# Autodesk Inventor assembly: wahacz_tylny_szkic
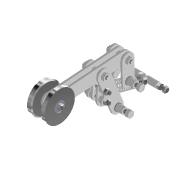
[picture p0: Inventor's stored thumbnail of the model, 180x180]
Saved by Autodesk Inventor 2020.3 (Build 243373000, 373)
## iProperties
Created: 2022-01-11
Part Number: wahacz_tylny_szkic
Document SubType Name: Assembly
Designer: patry
Author: patry
## Documents named in this file (27)
- C:\Users\patry\Desktop\Semestr 7\Inzynierka\Projekt inventor\Ariadna_inzynierka\Workspaces\Obszar roboczy\Obszar roboczy\Naped\Zawieszenie_v3\wahacz_tylny_szkic.iam
- C:\Users\patry\Desktop\Semestr 7\Inzynierka\Projekt inventor\Ariadna_inzynierka\Workspaces\Obszar roboczy\Obszar roboczy\Naped\Zawieszenie_v3\ramie_1_wahacza.ipt
- C:\Users\patry\Desktop\Semestr 7\Inzynierka\Projekt inventor\Ariadna_inzynierka\Workspaces\Obszar roboczy\Obszar roboczy\Naped\Zawieszenie_v3\tuleja_TUF106040.ipt
- C:\Users\patry\Desktop\Semestr 7\Inzynierka\Projekt inventor\Ariadna_inzynierka\Workspaces\Obszar roboczy\Obszar roboczy\Naped\Sruby\M6_nut_5mm.ipt
- C:\Users\patry\Desktop\Semestr 7\Inzynierka\Projekt inventor\Ariadna_inzynierka\Workspaces\Obszar roboczy\Obszar roboczy\Naped\Amortyzator\Korpus.ipt
- C:\Users\patry\Desktop\Semestr 7\Inzynierka\Projekt inventor\Ariadna_inzynierka\Workspaces\Obszar roboczy\Obszar roboczy\Naped\Amortyzator\Tlok.ipt
- C:\Users\patry\Desktop\Semestr 7\Inzynierka\Projekt inventor\Ariadna_inzynierka\Workspaces\Obszar roboczy\Obszar roboczy\Naped\Amortyzator\Nakretka.ipt
- C:\Users\patry\Desktop\Semestr 7\Inzynierka\Projekt inventor\Ariadna_inzynierka\Workspaces\Obszar roboczy\Obszar roboczy\Naped\Sruby\M5_nut_5mm.ipt
- C:\Users\patry\Desktop\Semestr 7\Inzynierka\Projekt inventor\Ariadna_inzynierka\Workspaces\Obszar roboczy\Obszar roboczy\Naped\Sruby\M5_70_shaft.ipt
- C:\Users\patry\Desktop\Semestr 7\Inzynierka\Projekt inventor\Ariadna_inzynierka\Workspaces\Obszar roboczy\Obszar roboczy\Naped\Sruby\M3_16_shaft.ipt
- C:\Users\patry\Desktop\Semestr 7\Inzynierka\Projekt inventor\Ariadna_inzynierka\Workspaces\Obszar roboczy\Obszar roboczy\Naped\Sruby\M3_nut_2,5mm.ipt
- C:\Users\patry\Desktop\Semestr 7\Inzynierka\Projekt inventor\Ariadna_inzynierka\Workspaces\Obszar roboczy\Obszar roboczy\Naped\Zawieszenie_v3\wspornik_amortyzatora.ipt
- C:\Users\patry\Desktop\Semestr 7\Inzynierka\Projekt inventor\Ariadna_inzynierka\Workspaces\Obszar roboczy\Obszar roboczy\Naped\Sruby\M6_40_shaft.ipt
- C:\Users\patry\Desktop\Semestr 7\Inzynierka\Projekt inventor\Ariadna_inzynierka\Workspaces\Obszar roboczy\Obszar roboczy\Naped\Sruby\tuleja_M6_M10_7.ipt
- C:\Users\patry\Desktop\Semestr 7\Inzynierka\Projekt inventor\Ariadna_inzynierka\Workspaces\Obszar roboczy\Obszar roboczy\Naped\Sruby\M6_1,25_pad.ipt
- C:\Users\patry\Desktop\Semestr 7\Inzynierka\Projekt inventor\Ariadna_inzynierka\Workspaces\Obszar roboczy\Obszar roboczy\Naped\Sruby\M6_70_shaft.ipt
- C:\Users\patry\Desktop\Semestr 7\Inzynierka\Projekt inventor\Ariadna_inzynierka\Workspaces\Obszar roboczy\Obszar roboczy\Naped\Sruby\M5_40_shaft.ipt
- M5_shaft.ipt
- C:\Users\patry\Desktop\Semestr 7\Inzynierka\Projekt inventor\Ariadna_inzynierka\Workspaces\Obszar roboczy\Obszar roboczy\Naped\Sruby\tuleja_M5_M9_4,5.ipt
- C:\Users\patry\Desktop\Semestr 7\Inzynierka\Projekt inventor\Ariadna_inzynierka\Workspaces\Obszar roboczy\Obszar roboczy\Naped\Zawieszenie_v3\glowny_wahacz_zewn.ipt
- lacznik_zewn.ipt
- C:\Users\patry\Desktop\Semestr 7\Inzynierka\Projekt inventor\Ariadna_inzynierka\Workspaces\Obszar roboczy\Obszar roboczy\Naped\Zawieszenie_v3\independent_wheel_pair.iam
- C:\Users\patry\Desktop\Semestr 7\Inzynierka\Projekt inventor\Ariadna_inzynierka\Workspaces\Obszar roboczy\Obszar roboczy\Naped\Sruby\tuleja_M6_M10_6.ipt
- C:\Users\patry\Desktop\Semestr 7\Inzynierka\Projekt inventor\Ariadna_inzynierka\Workspaces\Obszar roboczy\Obszar roboczy\Naped\Sruby\tuleja_M5_M9_17.5.ipt
- C:\Users\patry\Desktop\Semestr 7\Inzynierka\Projekt inventor\Ariadna_inzynierka\Workspaces\Obszar roboczy\Obszar roboczy\Naped\Zawieszenie_v3\ramie_2_wahacza_tylnego.ipt
- C:\Users\patry\Desktop\Semestr 7\Inzynierka\Projekt inventor\Ariadna_inzynierka\Workspaces\Obszar roboczy\Obszar roboczy\Naped\Sruby\M6x25_plaski_leb.ipt
- C:\Users\patry\Desktop\Semestr 7\Inzynierka\Projekt inventor\Ariadna_inzynierka\Workspaces\Obszar roboczy\Obszar roboczy\Naped\Zawieszenie_v3\Compress Spring11.ipt
## Components (73 placed, 24 different names)
1. ramie_1_wahacza:1
2. tuleja_TUF106040:1
3. tuleja_TUF106040:2
4. tuleja_TUF106040:3
5. tuleja_TUF106040:4
6. tuleja_TUF106040:5
7. tuleja_TUF106040:6
8. tuleja_TUF106040:7
9. tuleja_TUF106040:8
10. M6_nut_5mm:1
11. Korpus:1 — Zestawiające:139
12. Tlok:1 — Równoległe:10
13. Nakretka:1
14. M5_nut_5mm:1
15. M5_70_shaft:1
16. ramie_1_wahacza:2
17. M5_nut_5mm:2
18. M3_16_shaft:1
19. M3_nut_2,5mm:1
20. M3_nut_2,5mm:2
21. wspornik_amortyzatora:1
22. wspornik_amortyzatora:2
23. M6_40_shaft:1
24. M6_40_shaft:2
25. M6_nut_5mm:2
26. M6_nut_5mm:3
27. M6_nut_5mm:4
28. tuleja_M6_M10_7:1
29. tuleja_M6_M10_7:2
30. M6_1,25_pad:1
31. M6_1,25_pad:2
32. M6_1,25_pad:3
33. M6_1,25_pad:4
34. M6_1,25_pad:5
35. M6_1,25_pad:6
36. M6_1,25_pad:7
37. M6_1,25_pad:8
38. M6_70_shaft:1
39. M6_nut_5mm:5
40. M6_nut_5mm:6
41. M6_nut_5mm:7
42. M6_nut_5mm:8
43. M5_shaft:1
44. M5_shaft:2
45. M5_nut_5mm:3
46. M5_nut_5mm:4
47. M5_nut_5mm:5
48. M5_nut_5mm:6
49. tuleja_M5_M9_4,5:1
50. tuleja_M5_M9_4,5:2
51. tuleja_M5_M9_4,5:3
52. tuleja_M5_M9_4,5:4
53. lacznik_zewn:1
54. lacznik_zewn:2
55. independent_wheel_pair:1 [sub-assembly]
56. tuleja_M6_M10_7:3
57. tuleja_M6_M10_6:1
58. M6_nut_5mm:9
59. M6_nut_5mm:10
60. M6_nut_5mm:11
61. M6_nut_5mm:12
62. tuleja_M6_M10_6:2
63. tuleja_M6_M10_6:3
64. tuleja_M6_M10_6:4
65. M5_nut_5mm:7
66. M5_nut_5mm:8
67. tuleja_M5_M9_17.5:1
68. tuleja_M5_M9_17.5:2
69. ramie_2_wahacza_tylnego:1
70. ramie_2_wahacza_tylnego:2
71. M6x25_plaski_leb:1
72. M6x25_plaski_leb:2
73. Compress Spring1:1 — Zestawiające:139, Równoległe:10
## Relationships (152: Mate 139, Flush 10, Angle 2, CylindricalJoint 1)
- [Mate]: ramie_1_wahacza:1 ↔ tuleja_TUF106040:4
- [Mate]: ramie_1_wahacza:1 ↔ tuleja_TUF106040:4
- [Angle] (0 deg): ramie_1_wahacza:1 ↔ tuleja_TUF106040:4
- [Mate]: Korpus:1 ↔ Tlok:1
- [Angle] (0 deg): Korpus:1 ↔ Tlok:1
- [Mate]: Korpus:1 ↔ Nakretka:1
- [Mate] (10 mm): Korpus:1 ↔ Nakretka:1
- [CylindricalJoint]: Korpus:1 ↔ Tlok:1
- [Mate]: Korpus:1 ↔ M5_70_shaft:1
- [Flush] (-32.5 mm): Korpus:1 ↔ M5_70_shaft:1
- [Mate]: M5_nut_5mm:1 ↔ M5_70_shaft:1
- [Mate]: M5_70_shaft:1 ↔ M5_nut_5mm:2
- [Mate] (60 mm): M5_nut_5mm:1 ↔ M5_nut_5mm:2
- [Mate] (27.5 mm): Korpus:1 ↔ M5_nut_5mm:1
- [Mate]: tuleja_TUF106040:6 ↔ ramie_1_wahacza:2
- [Mate]: tuleja_TUF106040:5 ↔ ramie_1_wahacza:2
- [Mate]: tuleja_TUF106040:6 ↔ ramie_1_wahacza:2
- [Mate]: tuleja_TUF106040:1 ↔ tuleja_TUF106040:7
- [Mate]: wspornik_amortyzatora:1 ↔ wspornik_amortyzatora:2
- [Mate]: wspornik_amortyzatora:1 ↔ wspornik_amortyzatora:2
- [Mate] (5 mm): wspornik_amortyzatora:1 ↔ wspornik_amortyzatora:2
- [Mate]: M3_16_shaft:1 ↔ wspornik_amortyzatora:2
- [Flush] (-2.5 mm): M3_16_shaft:1 ↔ wspornik_amortyzatora:1
- [Mate]: M3_16_shaft:1 ↔ M3_nut_2,5mm:1
- [Mate]: M3_nut_2,5mm:1 ↔ wspornik_amortyzatora:1
- [Mate]: M3_16_shaft:1 ↔ M3_nut_2,5mm:2
- [Mate]: M3_nut_2,5mm:2 ↔ wspornik_amortyzatora:2
- [Mate]: Tlok:1 ↔ M3_16_shaft:1
- [Mate]: Tlok:1 ↔ wspornik_amortyzatora:2
- [Mate]: ramie_1_wahacza:1 ↔ wspornik_amortyzatora:1
- [Mate]: ramie_1_wahacza:1 ↔ wspornik_amortyzatora:1
- [Mate] (4.5 mm): ramie_1_wahacza:1 ↔ wspornik_amortyzatora:1
- [Mate]: tuleja_TUF106040:4 ↔ M6_40_shaft:1
- [Flush] (7 mm): ramie_1_wahacza:1 ↔ M6_40_shaft:1
- [Mate]: tuleja_TUF106040:7 ↔ M6_40_shaft:2
- [Mate]: M6_nut_5mm:1 ↔ M6_40_shaft:1
- [Mate]: ramie_1_wahacza:1 ↔ M6_nut_5mm:1
- [Mate]: M6_40_shaft:1 ↔ M6_nut_5mm:2
- [Mate]: ramie_1_wahacza:2 ↔ M6_nut_5mm:2
- [Mate]: M6_40_shaft:2 ↔ M6_nut_5mm:3
- [Mate]: M6_40_shaft:2 ↔ M6_nut_5mm:4
- [Mate]: M6_40_shaft:1 ↔ tuleja_M6_M10_7:1
- [Mate]: M6_40_shaft:2 ↔ tuleja_M6_M10_7:2
- [Mate]: M6_1,25_pad:1 ↔ M6_1,25_pad:2
- [Mate]: M6_1,25_pad:1 ↔ M6_1,25_pad:2
- [Mate]: M6_40_shaft:1 ↔ M6_1,25_pad:1
- [Mate]: M6_1,25_pad:3 ↔ M6_1,25_pad:4
- [Mate]: M6_1,25_pad:3 ↔ M6_1,25_pad:4
- [Mate]: M6_40_shaft:1 ↔ M6_1,25_pad:3
- [Mate]: tuleja_TUF106040:4 ↔ M6_1,25_pad:3
- [Mate]: M6_1,25_pad:5 ↔ M6_1,25_pad:6
- [Mate]: M6_1,25_pad:5 ↔ M6_1,25_pad:6
- [Mate]: M6_40_shaft:2 ↔ M6_1,25_pad:5
- [Mate]: M6_1,25_pad:7 ↔ M6_1,25_pad:8
- [Mate]: M6_1,25_pad:7 ↔ M6_1,25_pad:8
- [Mate]: M6_40_shaft:2 ↔ M6_1,25_pad:7
- [Mate]: tuleja_TUF106040:7 ↔ M6_1,25_pad:7
- [Flush]: M5_70_shaft:1 ↔ M6_70_shaft:1
- [Mate]: M6_70_shaft:1 ↔ M6_nut_5mm:5
- [Mate]: M6_70_shaft:1 ↔ M6_nut_5mm:6
- [Mate] (60 mm): M6_nut_5mm:5 ↔ M6_nut_5mm:6
- [Flush]: M5_nut_5mm:1 ↔ M6_nut_5mm:6
- [Mate] (60 mm): M6_nut_5mm:7 ↔ M6_nut_5mm:8
- [Mate]: M6_nut_5mm:7 ↔ M6_nut_5mm:8
- [Flush]: M5_nut_5mm:1 ↔ M6_nut_5mm:8
- [Mate]: ramie_1_wahacza:1 ↔ M5_shaft:1
- [Flush] (7 mm): ramie_1_wahacza:1 ↔ M5_shaft:1
- [Mate]: ramie_1_wahacza:1 ↔ M5_shaft:2
- [Flush] (7 mm): ramie_1_wahacza:1 ↔ M5_shaft:2
- [Mate]: M5_shaft:2 ↔ M5_nut_5mm:3
- [Mate]: ramie_1_wahacza:1 ↔ M5_nut_5mm:3
- [Mate]: M5_shaft:1 ↔ M5_nut_5mm:4
- [Mate]: ramie_1_wahacza:1 ↔ M5_nut_5mm:4
- [Mate]: M5_shaft:1 ↔ M5_nut_5mm:5
- [Mate]: ramie_1_wahacza:2 ↔ M5_nut_5mm:5
- [Mate]: M5_shaft:2 ↔ M5_nut_5mm:6
- [Mate]: ramie_1_wahacza:2 ↔ M5_nut_5mm:6
- [Mate]: M5_shaft:1 ↔ tuleja_M5_M9_4,5:1
- [Mate]: ramie_1_wahacza:2 ↔ tuleja_M5_M9_4,5:1
- [Mate]: M5_shaft:1 ↔ tuleja_M5_M9_4,5:2
- [Mate]: ramie_1_wahacza:1 ↔ tuleja_M5_M9_4,5:2
- [Mate]: M5_shaft:2 ↔ tuleja_M5_M9_4,5:3
- [Mate]: ramie_1_wahacza:2 ↔ tuleja_M5_M9_4,5:3
- [Mate]: M5_shaft:2 ↔ tuleja_M5_M9_4,5:4
- [Mate]: ramie_1_wahacza:1 ↔ tuleja_M5_M9_4,5:4
- [Mate]: M6_40_shaft:2 ↔ lacznik_zewn:1
- [Mate]: tuleja_M6_M10_7:2 ↔ lacznik_zewn:1
- [Mate]: M6_40_shaft:1 ↔ lacznik_zewn:1
- [Mate]: M6_40_shaft:2 ↔ lacznik_zewn:2
- [Mate]: M6_40_shaft:1 ↔ lacznik_zewn:2
- [Mate]: tuleja_TUF106040:6 ↔ M6_40_shaft:1
- [Mate]: M6_1,25_pad:4 ↔ lacznik_zewn:2
- [Mate]: M6_1,25_pad:8 ↔ lacznik_zewn:2
- [Mate]: tuleja_M6_M10_7:1 ↔ lacznik_zewn:1
- [Mate]: M6_1,25_pad:1 ↔ lacznik_zewn:1
- [Mate]: tuleja_TUF106040:6 ↔ M6_1,25_pad:2
- [Mate]: M6_1,25_pad:5 ↔ lacznik_zewn:1
- [Mate]: tuleja_TUF106040:1 ↔ M6_1,25_pad:6
- [Mate]: tuleja_TUF106040:5 ↔ ramie_1_wahacza:2
- [Mate]: tuleja_TUF106040:3 ↔ M6_70_shaft:1
- [Mate]: ramie_1_wahacza:1 ↔ tuleja_TUF106040:3
- [Mate]: ramie_1_wahacza:1 ↔ tuleja_TUF106040:3
- [Mate]: independent_wheel_pair:1 ↔ tuleja_M6_M10_7:3
- [Mate]: lacznik_zewn:2 ↔ independent_wheel_pair:1
- [Mate]: lacznik_zewn:2 ↔ independent_wheel_pair:1
- [Mate]: lacznik_zewn:2 ↔ tuleja_M6_M10_7:3
- [Mate]: ramie_1_wahacza:2 ↔ M5_shaft:2
- [Mate] (5 mm): M6_nut_5mm:8 ↔ M6_nut_5mm:9
- [Mate] (5 mm): M6_nut_5mm:7 ↔ M6_nut_5mm:10
- [Mate]: M6_70_shaft:1 ↔ M6_nut_5mm:11
- [Mate] (5 mm): M6_nut_5mm:5 ↔ M6_nut_5mm:11
- [Mate]: M6_70_shaft:1 ↔ M6_nut_5mm:12
- [Mate] (5 mm): M6_nut_5mm:6 ↔ M6_nut_5mm:12
- [Mate]: M6_70_shaft:1 ↔ tuleja_M6_M10_6:1
- [Mate]: tuleja_M6_M10_6:1 ↔ M6_nut_5mm:11
- [Mate]: tuleja_TUF106040:8 ↔ tuleja_M6_M10_6:2
- [Mate]: tuleja_TUF106040:2 ↔ tuleja_M6_M10_6:3
- [Mate]: M6_70_shaft:1 ↔ tuleja_M6_M10_6:4
- [Mate]: tuleja_TUF106040:5 ↔ tuleja_M6_M10_6:4
- [Mate]: M5_70_shaft:1 ↔ M5_nut_5mm:7
- [Mate] (5 mm): M5_nut_5mm:1 ↔ M5_nut_5mm:7
- [Mate]: M5_70_shaft:1 ↔ M5_nut_5mm:8
- [Mate] (5 mm): M5_nut_5mm:2 ↔ M5_nut_5mm:8
- [Mate]: M5_70_shaft:1 ↔ tuleja_M5_M9_17.5:2
- [Mate]: M5_nut_5mm:8 ↔ tuleja_M5_M9_17.5:2
- [Mate]: M5_70_shaft:1 ↔ tuleja_M5_M9_17.5:1
- [Mate]: Korpus:1 ↔ tuleja_M5_M9_17.5:1
- [Mate]: lacznik_zewn:1 ↔ independent_wheel_pair:1
- [Mate]: tuleja_TUF106040:1 ↔ ramie_2_wahacza_tylnego:1
- [Mate]: tuleja_TUF106040:1 ↔ ramie_2_wahacza_tylnego:1
- [Mate]: tuleja_TUF106040:2 ↔ ramie_2_wahacza_tylnego:1
- [Mate]: tuleja_TUF106040:2 ↔ ramie_2_wahacza_tylnego:1
- [Mate]: M6_nut_5mm:8 ↔ M6_nut_5mm:9
- [Mate] (5 mm): M6_nut_5mm:8 ↔ M6_nut_5mm:9
- [Mate]: M6_nut_5mm:9 ↔ tuleja_M6_M10_6:3
- [Mate]: tuleja_TUF106040:2 ↔ M6_nut_5mm:9
- [Mate]: tuleja_TUF106040:7 ↔ ramie_2_wahacza_tylnego:2
- [Mate]: tuleja_TUF106040:7 ↔ ramie_2_wahacza_tylnego:2
- [Mate]: tuleja_TUF106040:8 ↔ ramie_2_wahacza_tylnego:2
- [Mate]: tuleja_TUF106040:8 ↔ ramie_2_wahacza_tylnego:2
- [Mate]: tuleja_TUF106040:8 ↔ tuleja_M6_M10_6:2
- [Mate]: M6_nut_5mm:10 ↔ tuleja_M6_M10_6:2
- [Mate]: M6_nut_5mm:7 ↔ M6_nut_5mm:10
- [Mate]: M6_nut_5mm:10 ↔ M6x25_plaski_leb:2
- [Mate]: ramie_2_wahacza_tylnego:2 ↔ M6x25_plaski_leb:2
- [Mate]: tuleja_TUF106040:2 ↔ M6x25_plaski_leb:1
- [Mate]: ramie_2_wahacza_tylnego:1 ↔ M6x25_plaski_leb:1
- [Mate]: M6_nut_5mm:4 ↔ ramie_2_wahacza_tylnego:2
- [Mate]: M6_nut_5mm:3 ↔ ramie_2_wahacza_tylnego:1
- [Flush] (-2 mm): M6_40_shaft:2 ↔ M6_nut_5mm:3
- Zestawiające:139 [Mate]: Korpus:1 ↔ Compress Spring1:1
- Równoległe:10 [Flush]: Tlok:1 ↔ Compress Spring1:1
## Named parameters: d163_d155 = 0 mm, d166_d154 = 0 mm, d167_d155 = 0 mm, d178_d176 = 60 mm, d30_d120 = 0 mm, d31_d121 = 0 mm, d32_d122 = 5 mm, d33_d123 = 0 mm, d34_d124 = -2.5 mm, d35_d125 = 0 mm, d36_d126 = 0 mm, d37_d127 = 0 mm, d38_d128 = 0 mm, d39_d129 = 0 mm, d40_d130 = 0 mm, d41_d135 = 0 mm, d42_d136 = 0 mm, d43_d137 = 4.5 mm, d44_d138 = 0 mm, d45_d139 = 7 mm, d46_d140 = 0 mm, d47_d142 = 0 mm, d48_d143 = 0 mm, d49_d144 = 0 mm, d50_d145 = 0 mm, d51_d146 = 0 mm, d52_d148 = 0 mm, d53_d150 = 0 mm, d54_d152 = 0 mm, d55_d154 = 0 mm, d83_d6 = 0 mm, d84_d7 = -6.60527 mm, d85_d8 = -13 mm, d86_d0 = 0 mm, d87_d1 = 0 deg, d88_d3 = 0 mm, d89_d4 = 10 mm, d90_d5 = 0 deg, d66_d108 = 0 mm, d67_d109 = -32.5 mm, d68_d110 = 0 mm, d69_d111 = 0 mm, d70_d112 = 60 mm, d71_d113 = 27.5 mm, d72_d114 = 0 mm, d73_d115 = 0 mm, d74_d116 = 0 mm, d75_d119 = 0 mm, d2533_d208 = 0 mm, d2534_d209 = 0 mm, d158_d154 = 0 mm, d159_d155 = 0 mm, d162_d154 = 0 mm
